# Autodesk Inventor assembly: ROV Frame Assembly 1
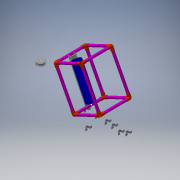
[picture p0: Inventor's stored thumbnail of the model, 180x180]
Saved by Autodesk Inventor 2016 (Build 200138000, 138)
## iProperties
Created: 2017-01-30
Part Number: ROV Frame Assembly 1
Document SubType Name: Assembly
Designer: Student
Author: Student
## Documents named in this file (11)
- C:\Users\Student\Desktop\Noah Code\ROV\ROV Frame Assembly 1.iam
- C:\Users\Student\Desktop\Noah Code\ROV\pvc pipe 1in 1.ipt
- C:\Users\Student\Desktop\Noah Code\ROV\pvc pipe 1in 3.ipt
- C:\Users\Student\Desktop\Noah Code\ROV\pvc pipe 1in 4.ipt
- C:\Users\Student\Desktop\Noah Code\ROV\pvc pipe 1in 1ft 1.ipt
- C:\Users\Student\Desktop\Noah Code\ROV\pvc pipe 1in 1ft 2.ipt
- C:\Users\Student\Desktop\ROV 2-2-17\pvc 1in 3 way elbow.ipt
- C:\Users\Student\Desktop\ROV 2-2-17\4 inch PVC pipe.ipt
- C:\Users\Student\Desktop\Noah Code\ROV\Attachy-thing Derek.ipt
- C:\Users\Student\Desktop\Noah Code\ROV\Control pipe holder V2.ipt
- C:\Users\Student\Desktop\ROV 2-2-17\O ring Dome 2.ipt
## Components (30 placed, 10 different names)
1. pvc pipe 1in 1:1 — Mate:24, Mate:25, Mate:28
2. pvc pipe 1in 3:1 — Cylindrical:1, Mate:4, Mate:13
3. pvc pipe 1in 4:1 — Mate:3, Mate:7, Mate:8, Mate:9
4. pvc pipe 1in 1ft 1:1 — Mate:14, Mate:15, Mate:34, Mate:35
5. pvc pipe 1in 1ft 2:1 — Mate:10, Mate:11, Mate:12
6. pvc pipe 1in 1ft 2:2 — Mate:16, Mate:17, Mate:29, Mate:30
7. pvc pipe 1in 1ft 2:3 — Mate:1, Mate:2, Mate:5, Mate:6
8. pvc 1in 3 way elbow:1 — Cylindrical:1, Mate:1, Mate:4, Mate:5, Mate:20, Mate:21
9. pvc 1in 3 way elbow:2 — Mate:2, Mate:3, Mate:6, Mate:7, Mate:16, Mate:17
10. pvc 1in 3 way elbow:3 — Mate:8, Mate:9, Mate:10, Mate:11, Mate:14, Mate:15
11. pvc 1in 3 way elbow:4 — Mate:12, Mate:13, Mate:18, Mate:19
12. pvc pipe 1in 1ft 1:2 — Mate:18, Mate:19, Mate:26, Mate:27
13. pvc pipe 1in 1ft 1:3 — Mate:20, Mate:21, Mate:22, Mate:23
14. pvc pipe 1in 1ft 1:4 — Mate:31, Mate:32, Mate:33
15. pvc pipe 1in 1ft 1:5 — Mate:36, Mate:37, Mate:38, Mate:39
16. pvc 1in 3 way elbow:5 — Mate:34, Mate:35, Mate:37, Mate:38, Mate:41
17. pvc 1in 3 way elbow:6 — Mate:29, Mate:30, Mate:33, Mate:40, Mate:42
18. pvc 1in 3 way elbow:7 — Mate:26, Mate:27, Mate:28, Mate:36, Mate:39
19. pvc 1in 3 way elbow:8 — Mate:22, Mate:23, Mate:24, Mate:25, Mate:31, Mate:32
20. pvc pipe 1in 3:2 — Mate:40, Mate:41, Mate:42
21. 4 inch PVC pipe:1
22. Attachy-thing Derek:1
23. Attachy-thing Derek:2
24. Attachy-thing Derek:3
25. Attachy-thing Derek:4
26. Attachy-thing Derek:5
27. Attachy-thing Derek:6
28. Attachy-thing Derek:7
29. Control pipe holder V2:1
30. O ring Dome 2:1
## Relationships (43: Mate 42, CylindricalJoint 1)
- Cylindrical:1: pvc pipe 1in 3:1 ↔ pvc 1in 3 way elbow:1
- Mate:1: pvc pipe 1in 1ft 2:3 ↔ pvc 1in 3 way elbow:1
- Mate:2: pvc pipe 1in 1ft 2:3 ↔ pvc 1in 3 way elbow:2
- Mate:3: pvc pipe 1in 4:1 ↔ pvc 1in 3 way elbow:2
- Mate:4: pvc pipe 1in 3:1 ↔ pvc 1in 3 way elbow:1
- Mate:5: pvc pipe 1in 1ft 2:3 ↔ pvc 1in 3 way elbow:1
- Mate:6: pvc pipe 1in 1ft 2:3 ↔ pvc 1in 3 way elbow:2
- Mate:7: pvc pipe 1in 4:1 ↔ pvc 1in 3 way elbow:2
- Mate:8: pvc pipe 1in 4:1 ↔ pvc 1in 3 way elbow:3
- Mate:9: pvc pipe 1in 4:1 ↔ pvc 1in 3 way elbow:3
- Mate:10: pvc pipe 1in 1ft 2:1 ↔ pvc 1in 3 way elbow:3
- Mate:11: pvc pipe 1in 1ft 2:1 ↔ pvc 1in 3 way elbow:3
- Mate:12: pvc pipe 1in 1ft 2:1 ↔ pvc 1in 3 way elbow:4
- Mate:13: pvc pipe 1in 3:1 ↔ pvc 1in 3 way elbow:4
- Mate:14: pvc pipe 1in 1ft 1:1 ↔ pvc 1in 3 way elbow:3
- Mate:15: pvc pipe 1in 1ft 1:1 ↔ pvc 1in 3 way elbow:3
- Mate:16: pvc pipe 1in 1ft 2:2 ↔ pvc 1in 3 way elbow:2
- Mate:17: pvc pipe 1in 1ft 2:2 ↔ pvc 1in 3 way elbow:2
- Mate:18: pvc 1in 3 way elbow:4 ↔ pvc pipe 1in 1ft 1:2
- Mate:19: pvc 1in 3 way elbow:4 ↔ pvc pipe 1in 1ft 1:2
- Mate:20: pvc 1in 3 way elbow:1 ↔ pvc pipe 1in 1ft 1:3
- Mate:21: pvc 1in 3 way elbow:1 ↔ pvc pipe 1in 1ft 1:3
- Mate:22: pvc pipe 1in 1ft 1:3 ↔ pvc 1in 3 way elbow:8
- Mate:23: pvc pipe 1in 1ft 1:3 ↔ pvc 1in 3 way elbow:8
- Mate:24: pvc pipe 1in 1:1 ↔ pvc 1in 3 way elbow:8
- Mate:25: pvc pipe 1in 1:1 ↔ pvc 1in 3 way elbow:8
- Mate:26: pvc pipe 1in 1ft 1:2 ↔ pvc 1in 3 way elbow:7
- Mate:27: pvc pipe 1in 1ft 1:2 ↔ pvc 1in 3 way elbow:7
- Mate:28: pvc pipe 1in 1:1 ↔ pvc 1in 3 way elbow:7
- Mate:29: pvc pipe 1in 1ft 2:2 ↔ pvc 1in 3 way elbow:6
- Mate:30: pvc pipe 1in 1ft 2:2 ↔ pvc 1in 3 way elbow:6
- Mate:31: pvc pipe 1in 1ft 1:4 ↔ pvc 1in 3 way elbow:8
- Mate:32: pvc pipe 1in 1ft 1:4 ↔ pvc 1in 3 way elbow:8
- Mate:33: pvc pipe 1in 1ft 1:4 ↔ pvc 1in 3 way elbow:6
- Mate:34: pvc pipe 1in 1ft 1:1 ↔ pvc 1in 3 way elbow:5
- Mate:35: pvc pipe 1in 1ft 1:1 ↔ pvc 1in 3 way elbow:5
- Mate:36: pvc pipe 1in 1ft 1:5 ↔ pvc 1in 3 way elbow:7
- Mate:37: pvc pipe 1in 1ft 1:5 ↔ pvc 1in 3 way elbow:5
- Mate:38: pvc pipe 1in 1ft 1:5 ↔ pvc 1in 3 way elbow:5
- Mate:39: pvc pipe 1in 1ft 1:5 ↔ pvc 1in 3 way elbow:7
- Mate:40: pvc 1in 3 way elbow:6 ↔ pvc pipe 1in 3:2
- Mate:41: pvc 1in 3 way elbow:5 ↔ pvc pipe 1in 3:2
- Mate:42: pvc 1in 3 way elbow:6 ↔ pvc pipe 1in 3:2
